# Autodesk Inventor assembly: Mass 2
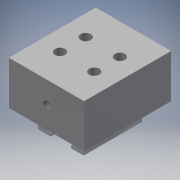
[picture p0: Inventor's stored thumbnail of the model, 180x180]
Saved by Autodesk Inventor 2016 (Build 200138000, 138)
## iProperties
Created: 2015-06-08
Part Number: Mass 2
Document SubType Name: Assembly
Designer: Dennis
Author: Dennis
## Documents named in this file (3)
- C:\Users\Dennis\Dropbox\NI Work\NI Slider Crank\Assemblies\Mass 2.iam
- C:\Users\Dennis\Dropbox\NI Work\NI Slider Crank\Parts\Carriage - 9829K300.ipt
- C:\Users\Dennis\Dropbox\NI Work\NI Slider Crank\Parts\Mass 2.ipt
## Components (2 placed, 2 different names)
1. Carriage - 9829K300:1 — Mate:1, Mate:2, Mate:3
2. Mass 2:1 — Mate:1, Mate:2, Mate:3
## Relationships (3: Mate 3)
- Mate:1: Carriage - 9829K300:1 ↔ Mass 2:1
- Mate:2: Carriage - 9829K300:1 ↔ Mass 2:1
- Mate:3: Carriage - 9829K300:1 ↔ Mass 2:1
